# Autodesk Inventor assembly: motor
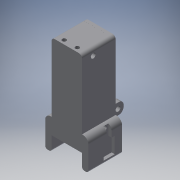
[picture p0: Inventor's stored thumbnail of the model, 180x180]
Saved by Autodesk Inventor 2016 (Build 200138000, 138)
## iProperties
Created: 2016-11-21
Part Number: motor
Document SubType Name: Assembly
Designer: Juraj
Author: Juraj
## Documents named in this file (3)
- C:\Users\Juraj\Documents\GitHub\Robot6x6\Terrenny robot CAD\uchyt_motor\motor.iam
- C:\Users\Juraj\Documents\GitHub\Robot6x6\Terrenny robot CAD\uchyt_motor\Part1.ipt
- C:\Users\Juraj\Documents\GitHub\Robot6x6\Terrenny robot CAD\uchyt_motor\Part2.ipt
## Components (2 placed, 2 different names)
1. Part1:1 — Insert:1, Insert:2
2. Part2:1 — Insert:1, Insert:2
## Relationships (2: Insert 2)
- Insert:1: Part1:1 ↔ Part2:1
- Insert:2: Part1:1 ↔ Part2:1
